# Autodesk Inventor assembly: Turntable Outer Gear
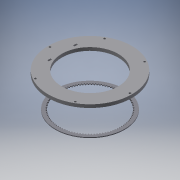
[picture p0: Inventor's stored thumbnail of the model, 180x180]
Saved by Autodesk Inventor 2016 (Build 200138000, 138)
## iProperties
Created: 2016-04-25
Part Number: Turntable Outer Gear
Document SubType Name: Assembly
Designer: rubenjm
Author: rubenjm
## Documents named in this file (3)
- C:\Users\rubenjm\Documents\To Transfer\2k16 Spring\RME\GGC\V3\Turntable Outer Gear.iam
- C:\Users\rubenjm\Documents\To Transfer\2k16 Spring\RME\GGC\V3\Turntable Outer Gear.ipt
- C:\Users\rubenjm\Documents\To Transfer\2k16 Spring\RME\GGC\V3\Turntable Outer Gear\Design Accelerator\Spur Gears2.iam
## Components (2 placed, 2 different names)
1. Turntable Outer Gear:1 — Mate:1, Mate:2
2. Spur Gears:2 [sub-assembly] — Mate:1, Mate:2
## Relationships (2: Mate 2)
- Mate:1: Turntable Outer Gear:1 ↔ Spur Gears:2
- Mate:2: Turntable Outer Gear:1 ↔ Spur Gears:2
